# Autodesk Inventor assembly: ADSK-MH-10027
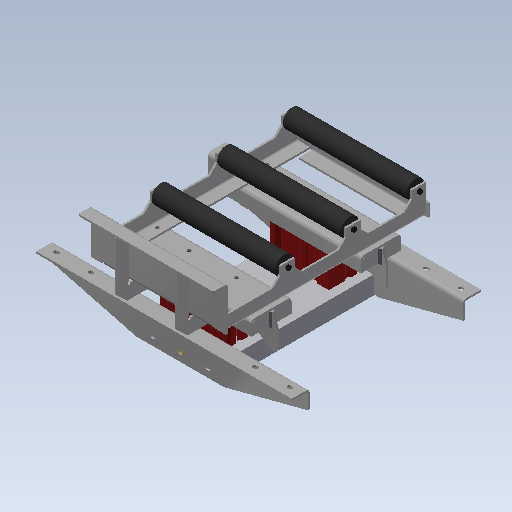
[picture p0: Inventor's stored thumbnail of the model, 512x512]
Saved by Autodesk Inventor 2020.2 (Build 242310000, 310)
## iProperties
Created: 2008-03-12
Part Number: ADSK-MH-10027
Document SubType Name: Assembly
Designer: R.O'mahony
Description: Discharge Platform Assembly
Engineer: Demir Ali
Checked By: Demir Ali
Company: Autodesk Ltd
Author: R.O'mahony
Keywords: Roller Conveyor
Revision Number: A
## Documents named in this file (4)
- C:\Users\peter\source\repos\InventorDA-FLC\Dataset\Discharge Conveyor\ADSK-MH-10027.iam
- C:\Users\peter\source\repos\InventorDA-FLC\Dataset\Discharge Conveyor\ADSK-MH-10024.iam
- C:\Users\peter\source\repos\InventorDA-FLC\Dataset\Discharge Conveyor\ADSK-MH-10028.iam
- C:\Users\peter\source\repos\InventorDA-FLC\Dataset\Discharge Conveyor\ADSK-MH-10031.iam
## Components (4 placed, 3 different names)
1. ADSK-MH-10024:2 [sub-assembly] — Mate:21, Mate:22, Mate:23
2. ADSK-MH-10031:1 [sub-assembly] — Rigid:1
3. ADSK-MH-10028:1 [sub-assembly] — Mate:21, Mate:22, Mate:23, Rigid:1
4. ADSK-MH-10028:2 [sub-assembly]
## Component patterns: (2 elements, first: ADSK-MH-10028:1)
## Relationships (4: Mate 3, WeldJoint 1)
- Mate:21: ADSK-MH-10024:2 ↔ ADSK-MH-10028:1
- Mate:22: ADSK-MH-10024:2 ↔ ADSK-MH-10028:1
- Mate:23: ADSK-MH-10024:2 ↔ ADSK-MH-10028:1
- Rigid:1 [WeldJoint]: ADSK-MH-10031:1 ↔ ADSK-MH-10028:1
